# Autodesk Inventor assembly: Final Assembly
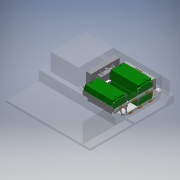
[picture p0: Inventor's stored thumbnail of the model, 180x180]
Saved by Autodesk Inventor 2017 (Build 210142000, 142)
## iProperties
Created: 2022-08-16
Part Number: Final Assembly
Document SubType Name: Assembly
Designer: JTS
Author: JTS
## Documents named in this file (24)
- G:\47 Ah FoMoCo Tray\02 Final Assembly (Tray Mated).iam
- G:\47 Ah FoMoCo Tray\LiBCM003 - Battery Tray\47 Ah FoMoCo Aluminum Tray.ipt
- G:\47 Ah FoMoCo Tray\OEM Parts\Junction Board.ipt
- G:\47 Ah FoMoCo Tray\OEM Parts\MCM.ipt
- G:\47 Ah FoMoCo Tray\Battery Modules\47Ah-FoMoCo.ipt
- G:\47 Ah FoMoCo Tray\LiBCM004 - Battery Rail\Bracket - 5th Module 8982K875.ipt
- G:\47 Ah FoMoCo Tray\Nuts & Bolts\Ring Terminal.ipt
- G:\47 Ah FoMoCo Tray\Final Assembly\AIP\Cable and Harness\Final Assembly.Harness2.iam
- G:\47 Ah FoMoCo Tray\LiBCM PCB\LiBCM Safety Cover - RevC.ipt
- G:\47 Ah FoMoCo Tray\LiBCM PCB\PCB.ipt
- G:\47 Ah FoMoCo Tray\OEM Parts\IMA Bay - Battery Enclosure Interface.ipt
- G:\47 Ah FoMoCo Tray\Nuts & Bolts\Battery Bolt.iam
- G:\47 Ah FoMoCo Tray\Nuts & Bolts\Threaded Standoff.ipt
- G:\47 Ah FoMoCo Tray\Nuts & Bolts\Battery Bolt - Split Washer.iam
- G:\47 Ah FoMoCo Tray\Nuts & Bolts\Washer 0.250in 92141A029.ipt
- G:\47 Ah FoMoCo Tray\Nuts & Bolts\Nut - Hex - 0.250in-20 91845A029.ipt
- G:\47 Ah FoMoCo Tray\Nuts & Bolts\Top Spacer.ipt
- G:\47 Ah FoMoCo Tray\Nuts & Bolts\PEMSERT.ipt
- G:\47 Ah FoMoCo Tray\Grid Chargers\UHP-1500-230.ipt
- G:\47 Ah FoMoCo Tray\Grid Chargers\HLG-480H-C2100B.ipt
- G:\47 Ah FoMoCo Tray\LiBCM005 - Charger Mount\Charger Mount.ipt
- G:\47 Ah FoMoCo Tray\Grid Chargers\HLG-240H-C1050B.ipt
- G:\47 Ah FoMoCo Tray\Nuts & Bolts\Fan.ipt
- G:\47 Ah FoMoCo Tray\Nuts & Bolts\Power Resistor - HSA25.ipt
## Components (86 placed, 23 different names)
1. IMA Bay - Battery Enclosure Interface:1 — Insert:56, Mate:2, Mate:3, Mate:4
2. Junction Board:1 — Insert:11, Insert:12
3. MCM:1 — Insert:137, Insert:138
4. Harness2 [sub-assembly]
5. Washer 0.250in 92141A029:3 — Insert:124
6. Nut - Hex - 0.250in-20 91845A029:5
7. Top Spacer:1 — Insert:125, Insert:126
8. PEMSERT:1 — Insert:129
9. PEMSERT:2 — Insert:130
10. PEMSERT:3 — Insert:131
11. PEMSERT:4 — Insert:132
12. UHP-1500-230:1 — Mate:5, Mate:6, Flush:2, Flush:8, Flush:9
13. HLG-240H-C1050B:1 — Mate:8, Flush:10, Flush:11
14. HLG-480H-C2100B:1 — Mate:7, Flush:8, Flush:9, Flush:10, Flush:11
15. Charger Mount:1 — Flush:5, Flush:6, Mate:8, Insert:133, Insert:134
16. Fan:1 — Insert:133, Insert:134
17. Power Resistor - HSA25:15 — Mate:9, Mate:10, Flush:16
18. Power Resistor - HSA25:11 — Mate:11, Flush:12, Flush:31
19. Power Resistor - HSA25:9 — Mate:12, Flush:27, Flush:28
20. Power Resistor - HSA25:12 — Mate:21, Flush:20
21. Power Resistor - HSA25:3 — Mate:23
22. Power Resistor - HSA25:10 — Mate:15, Flush:30, Flush:31
23. Power Resistor - HSA25:16 — Mate:16, Flush:16, Flush:17
24. Power Resistor - HSA25:17 — Mate:17, Flush:17, Flush:18
25. Power Resistor - HSA25:18 — Mate:18, Flush:18
26. Power Resistor - HSA25:13 — Mate:19, Mate:34, Mate:35
27. Power Resistor - HSA25:2 — Mate:24, Flush:23
28. Power Resistor - HSA25:5 — Mate:26, Flush:24
29. Power Resistor - HSA25:6 — Mate:32, Flush:24, Flush:25
30. Power Resistor - HSA25:4 — Mate:27, Flush:25
31. Power Resistor - HSA25:8 — Mate:28, Flush:26, Flush:27
32. Power Resistor - HSA25:7 — Mate:30, Mate:36, Flush:26
33. Power Resistor - HSA25:14 — Mate:31, Flush:29
34. Power Resistor - HSA25:1 — Mate:33, Flush:22
35. Power Resistor - HSA25:19 — Mate:37, Flush:28
36. Top Spacer:2 — Insert:135, Insert:138
37. Top Spacer:3 — Insert:136, Insert:137
38. Power Resistor - HSA25:20 — Mate:38, Flush:30
39. 47 Ah FoMoCo Aluminum Tray:1 — Insert:11, Insert:12, Insert:56, Mate:2, Insert:97, Insert:98, Insert:99, Insert:100, Insert:101, Insert:102, Insert:103, Insert:104, Insert:105, Insert:106, Insert:107, Insert:108, Insert:124, Mate:9, Mate:10, Mate:11, Flush:12, Mate:12, Mate:15, Mate:16, Mate:17, Mate:18, Mate:26, Mate:27, Mate:28, Mate:30, Mate:32, Mate:36, Mate:37, Insert:135, Insert:136, Mate:38
40. LiBCM Safety Cover - RevC:1 — Insert:55, Mate:1, Mate:3, Flush:1, Mate:4
41. PCB:1 — Insert:55, Mate:1
42. Threaded Standoff:1 — Insert:65
43. Threaded Standoff:2 — Insert:70
44. Threaded Standoff:3 — Insert:71
45. Threaded Standoff:4 — Insert:72, Insert:114
46. Threaded Standoff:5 — Insert:69, Insert:113
47. Threaded Standoff:6 — Insert:68, Insert:110
48. Threaded Standoff:7 — Insert:67
49. Threaded Standoff:8 — Insert:66, Insert:109
50. Battery Bolt:1 [sub-assembly] — Insert:102
51. Battery Bolt:2 [sub-assembly] — Insert:101
52. Battery Bolt:3 [sub-assembly] — Insert:99
53. Battery Bolt:4 [sub-assembly] — Insert:98
54. Battery Bolt:5 [sub-assembly] — Insert:100
55. Battery Bolt:6 [sub-assembly] — Insert:104
56. Battery Bolt:7 [sub-assembly] — Insert:103
57. Battery Bolt:8 [sub-assembly] — Insert:97
58. 47Ah-FoMoCo:1 — Insert:41, Insert:43, Tangent:1, Tangent:7, Insert:65, Insert:66, Insert:71, Insert:72, Insert:107, Insert:108
59. 47Ah-FoMoCo:2 — Insert:42, Insert:44, Tangent:3, Tangent:13, Insert:67, Insert:68, Insert:69, Insert:70, Insert:105, Insert:106
60. Bracket - 5th Module 8982K875:1 — Insert:109, Insert:110, Insert:120, Insert:121, Insert:122, Insert:131, Insert:132, Mate:5, Mate:6, Flush:2, Mate:7, Mate:19, Mate:21, Mate:31, Flush:20, Mate:34, Mate:35, Flush:29
61. Bracket - 5th Module 8982K875:2 — Insert:113, Insert:114, Insert:117, Insert:118, Insert:119, Insert:129, Insert:130, Flush:5, Flush:6, Mate:23, Mate:24, Mate:33, Flush:22, Flush:23
62. Battery Bolt:9 [sub-assembly] — Insert:127
63. Battery Bolt:10 [sub-assembly] — Insert:128
64. Battery Bolt - Split Washer:1 [sub-assembly] — Insert:77
65. Battery Bolt - Split Washer:2 [sub-assembly] — Insert:78
66. Battery Bolt - Split Washer:3 [sub-assembly] — Insert:79
67. Battery Bolt - Split Washer:4 [sub-assembly] — Insert:80
68. Battery Bolt - Split Washer:5 [sub-assembly] — Insert:84
69. Battery Bolt - Split Washer:6 [sub-assembly] — Insert:83
70. Battery Bolt - Split Washer:7 [sub-assembly] — Insert:82
71. Battery Bolt - Split Washer:8 [sub-assembly] — Insert:81
72. Battery Bolt - Split Washer:9 [sub-assembly] — Insert:126
73. Battery Bolt - Split Washer:10 [sub-assembly] — Insert:85
74. 47Ah-FoMoCo:3 — Insert:37, Insert:40, Tangent:9, Tangent:12, Flush:1, Insert:79, Insert:80, Insert:81, Insert:82, Insert:121, Insert:122
75. 47Ah-FoMoCo:4 — Insert:36, Insert:39, Tangent:14, Tangent:15, Insert:77, Insert:78, Insert:83, Insert:84, Insert:119, Insert:120
76. 47Ah-FoMoCo:5 — Insert:35, Insert:38, Tangent:16, Tangent:17, Insert:85, Insert:117, Insert:118, Insert:125, Insert:127, Insert:128
77. Ring Terminal:1 — Insert:35, Tangent:16
78. Ring Terminal:2 — Insert:36, Tangent:15
79. Ring Terminal:3 — Insert:37, Tangent:9
80. Ring Terminal:4 — Insert:38, Tangent:17
81. Ring Terminal:5 — Insert:39, Tangent:14
82. Ring Terminal:6 — Insert:40, Tangent:12
83. Ring Terminal:7 — Insert:41, Tangent:1
84. Ring Terminal:8 — Insert:42, Tangent:13
85. Ring Terminal:9 — Insert:43, Tangent:7
86. Ring Terminal:10 — Insert:44, Tangent:3
## Relationships (134: Insert 69, Mate 32, Flush 23, Tangent 10)
- Insert:11: Junction Board:1 ↔ 47 Ah FoMoCo Aluminum Tray:1
- Insert:12: Junction Board:1 ↔ 47 Ah FoMoCo Aluminum Tray:1
- Insert:35: 47Ah-FoMoCo:5 ↔ Ring Terminal:1
- Insert:36: 47Ah-FoMoCo:4 ↔ Ring Terminal:2
- Insert:37: 47Ah-FoMoCo:3 ↔ Ring Terminal:3
- Insert:38: 47Ah-FoMoCo:5 ↔ Ring Terminal:4
- Insert:39: 47Ah-FoMoCo:4 ↔ Ring Terminal:5
- Insert:40: 47Ah-FoMoCo:3 ↔ Ring Terminal:6
- Insert:41: 47Ah-FoMoCo:1 ↔ Ring Terminal:7
- Insert:42: 47Ah-FoMoCo:2 ↔ Ring Terminal:8
- Insert:43: 47Ah-FoMoCo:1 ↔ Ring Terminal:9
- Insert:44: 47Ah-FoMoCo:2 ↔ Ring Terminal:10
- Tangent:1 (2 mm): 47Ah-FoMoCo:1 ↔ Ring Terminal:7
- Tangent:3 (4 mm): 47Ah-FoMoCo:2 ↔ Ring Terminal:10
- Tangent:7 (6 mm): 47Ah-FoMoCo:1 ↔ Ring Terminal:9
- Tangent:9 (2 mm): 47Ah-FoMoCo:3 ↔ Ring Terminal:3
- Tangent:12 (2 mm): 47Ah-FoMoCo:3 ↔ Ring Terminal:6
- Tangent:13 (2 mm): 47Ah-FoMoCo:2 ↔ Ring Terminal:8
- Tangent:14 (2 mm): 47Ah-FoMoCo:4 ↔ Ring Terminal:5
- Tangent:15 (2 mm): 47Ah-FoMoCo:4 ↔ Ring Terminal:2
- Tangent:16 (2 mm): 47Ah-FoMoCo:5 ↔ Ring Terminal:1
- Tangent:17 (2 mm): 47Ah-FoMoCo:5 ↔ Ring Terminal:4
- Insert:55 (37 mm): LiBCM Safety Cover - RevC:1 ↔ PCB:1
- Mate:1: LiBCM Safety Cover - RevC:1 ↔ PCB:1
- Insert:56: IMA Bay - Battery Enclosure Interface:1 ↔ 47 Ah FoMoCo Aluminum Tray:1
- Mate:2: IMA Bay - Battery Enclosure Interface:1 ↔ 47 Ah FoMoCo Aluminum Tray:1
- Mate:3 (5 mm): IMA Bay - Battery Enclosure Interface:1 ↔ LiBCM Safety Cover - RevC:1
- Flush:1 (45 mm): LiBCM Safety Cover - RevC:1 ↔ 47Ah-FoMoCo:3
- Mate:4 (31.5 mm): IMA Bay - Battery Enclosure Interface:1 ↔ LiBCM Safety Cover - RevC:1
- Insert:65: Threaded Standoff:1 ↔ 47Ah-FoMoCo:1
- Insert:66: Threaded Standoff:8 ↔ 47Ah-FoMoCo:1
- Insert:67: Threaded Standoff:7 ↔ 47Ah-FoMoCo:2
- Insert:68: Threaded Standoff:6 ↔ 47Ah-FoMoCo:2
- Insert:69: Threaded Standoff:5 ↔ 47Ah-FoMoCo:2
- Insert:70: Threaded Standoff:2 ↔ 47Ah-FoMoCo:2
- Insert:71: Threaded Standoff:3 ↔ 47Ah-FoMoCo:1
- Insert:72: Threaded Standoff:4 ↔ 47Ah-FoMoCo:1
- Insert:77: Battery Bolt - Split Washer:1 ↔ 47Ah-FoMoCo:4
- Insert:78: Battery Bolt - Split Washer:2 ↔ 47Ah-FoMoCo:4
- Insert:79: Battery Bolt - Split Washer:3 ↔ 47Ah-FoMoCo:3
- Insert:80: Battery Bolt - Split Washer:4 ↔ 47Ah-FoMoCo:3
- Insert:81: Battery Bolt - Split Washer:8 ↔ 47Ah-FoMoCo:3
- Insert:82: Battery Bolt - Split Washer:7 ↔ 47Ah-FoMoCo:3
- Insert:83: Battery Bolt - Split Washer:6 ↔ 47Ah-FoMoCo:4
- Insert:84: Battery Bolt - Split Washer:5 ↔ 47Ah-FoMoCo:4
- Insert:85: Battery Bolt - Split Washer:10 ↔ 47Ah-FoMoCo:5
- Insert:97: 47 Ah FoMoCo Aluminum Tray:1 ↔ Battery Bolt:8
- Insert:98: 47 Ah FoMoCo Aluminum Tray:1 ↔ Battery Bolt:4
- Insert:99: 47 Ah FoMoCo Aluminum Tray:1 ↔ Battery Bolt:3
- Insert:100: 47 Ah FoMoCo Aluminum Tray:1 ↔ Battery Bolt:5
- Insert:101: 47 Ah FoMoCo Aluminum Tray:1 ↔ Battery Bolt:2
- Insert:102: 47 Ah FoMoCo Aluminum Tray:1 ↔ Battery Bolt:1
- Insert:103: 47 Ah FoMoCo Aluminum Tray:1 ↔ Battery Bolt:7
- Insert:104: 47 Ah FoMoCo Aluminum Tray:1 ↔ Battery Bolt:6
- Insert:105: 47 Ah FoMoCo Aluminum Tray:1 ↔ 47Ah-FoMoCo:2
- Insert:106: 47 Ah FoMoCo Aluminum Tray:1 ↔ 47Ah-FoMoCo:2
- Insert:107: 47 Ah FoMoCo Aluminum Tray:1 ↔ 47Ah-FoMoCo:1
- Insert:108: 47 Ah FoMoCo Aluminum Tray:1 ↔ 47Ah-FoMoCo:1
- Insert:109: Threaded Standoff:8 ↔ Bracket - 5th Module 8982K875:1
- Insert:110: Threaded Standoff:6 ↔ Bracket - 5th Module 8982K875:1
- Insert:113: Threaded Standoff:5 ↔ Bracket - 5th Module 8982K875:2
- Insert:114: Threaded Standoff:4 ↔ Bracket - 5th Module 8982K875:2
- Insert:117: Bracket - 5th Module 8982K875:2 ↔ 47Ah-FoMoCo:5
- Insert:118: Bracket - 5th Module 8982K875:2 ↔ 47Ah-FoMoCo:5
- Insert:119: Bracket - 5th Module 8982K875:2 ↔ 47Ah-FoMoCo:4
- Insert:120: Bracket - 5th Module 8982K875:1 ↔ 47Ah-FoMoCo:4
- Insert:121: Bracket - 5th Module 8982K875:1 ↔ 47Ah-FoMoCo:3
- Insert:122: Bracket - 5th Module 8982K875:1 ↔ 47Ah-FoMoCo:3
- [Insert]: Washer 0.250in 92141A029:3 ↔ Nut - Hex - 0.250in-20 91845A029:5
- Insert:124: Washer 0.250in 92141A029:3 ↔ 47 Ah FoMoCo Aluminum Tray:1
- Insert:125: Top Spacer:1 ↔ 47Ah-FoMoCo:5
- Insert:126: Top Spacer:1 ↔ Battery Bolt - Split Washer:9
- Insert:127: Battery Bolt:9 ↔ 47Ah-FoMoCo:5
- Insert:128: Battery Bolt:10 ↔ 47Ah-FoMoCo:5
- Insert:129: PEMSERT:1 ↔ Bracket - 5th Module 8982K875:2
- Insert:130: PEMSERT:2 ↔ Bracket - 5th Module 8982K875:2
- Insert:131: PEMSERT:3 ↔ Bracket - 5th Module 8982K875:1
- Insert:132: PEMSERT:4 ↔ Bracket - 5th Module 8982K875:1
- Mate:5: UHP-1500-230:1 ↔ Bracket - 5th Module 8982K875:1
- Mate:6 (1 mm): UHP-1500-230:1 ↔ Bracket - 5th Module 8982K875:1
- Flush:2: UHP-1500-230:1 ↔ Bracket - 5th Module 8982K875:1
- Mate:7: HLG-480H-C2100B:1 ↔ Bracket - 5th Module 8982K875:1
- Flush:5: Charger Mount:1 ↔ Bracket - 5th Module 8982K875:2
- Flush:6: Charger Mount:1 ↔ Bracket - 5th Module 8982K875:2
- Mate:8: HLG-240H-C1050B:1 ↔ Charger Mount:1
- Flush:8: UHP-1500-230:1 ↔ HLG-480H-C2100B:1
- Flush:9: UHP-1500-230:1 ↔ HLG-480H-C2100B:1
- Flush:10: HLG-240H-C1050B:1 ↔ HLG-480H-C2100B:1
- Flush:11: HLG-240H-C1050B:1 ↔ HLG-480H-C2100B:1
- Insert:133: Charger Mount:1 ↔ Fan:1
- Insert:134: Charger Mount:1 ↔ Fan:1
- Mate:9: Power Resistor - HSA25:15 ↔ 47 Ah FoMoCo Aluminum Tray:1
- Mate:10 (2.5 mm): Power Resistor - HSA25:15 ↔ 47 Ah FoMoCo Aluminum Tray:1
- Mate:11: Power Resistor - HSA25:11 ↔ 47 Ah FoMoCo Aluminum Tray:1
- Flush:12: Power Resistor - HSA25:11 ↔ 47 Ah FoMoCo Aluminum Tray:1
- Mate:12: Power Resistor - HSA25:9 ↔ 47 Ah FoMoCo Aluminum Tray:1
- Mate:15: Power Resistor - HSA25:10 ↔ 47 Ah FoMoCo Aluminum Tray:1
- Mate:16: Power Resistor - HSA25:16 ↔ 47 Ah FoMoCo Aluminum Tray:1
- Flush:16: Power Resistor - HSA25:15 ↔ Power Resistor - HSA25:16
- Mate:17: Power Resistor - HSA25:17 ↔ 47 Ah FoMoCo Aluminum Tray:1
- Flush:17: Power Resistor - HSA25:16 ↔ Power Resistor - HSA25:17
- Mate:18: Power Resistor - HSA25:18 ↔ 47 Ah FoMoCo Aluminum Tray:1
- Flush:18: Power Resistor - HSA25:17 ↔ Power Resistor - HSA25:18
- Mate:19: Power Resistor - HSA25:13 ↔ Bracket - 5th Module 8982K875:1
- Mate:21: Power Resistor - HSA25:12 ↔ Bracket - 5th Module 8982K875:1
- Mate:23: Power Resistor - HSA25:3 ↔ Bracket - 5th Module 8982K875:2
- Mate:24: Power Resistor - HSA25:2 ↔ Bracket - 5th Module 8982K875:2
- Mate:26: Power Resistor - HSA25:5 ↔ 47 Ah FoMoCo Aluminum Tray:1
- Mate:27: Power Resistor - HSA25:4 ↔ 47 Ah FoMoCo Aluminum Tray:1
- Mate:28: Power Resistor - HSA25:8 ↔ 47 Ah FoMoCo Aluminum Tray:1
- Mate:30: Power Resistor - HSA25:7 ↔ 47 Ah FoMoCo Aluminum Tray:1
- Mate:31: Power Resistor - HSA25:14 ↔ Bracket - 5th Module 8982K875:1
- Mate:32: Power Resistor - HSA25:6 ↔ 47 Ah FoMoCo Aluminum Tray:1
- Mate:33: Power Resistor - HSA25:1 ↔ Bracket - 5th Module 8982K875:2
- Flush:20: Power Resistor - HSA25:12 ↔ Bracket - 5th Module 8982K875:1
- Mate:34: Power Resistor - HSA25:13 ↔ Bracket - 5th Module 8982K875:1
- Mate:35: Power Resistor - HSA25:13 ↔ Bracket - 5th Module 8982K875:1
- Flush:22: Power Resistor - HSA25:1 ↔ Bracket - 5th Module 8982K875:2
- Flush:23: Power Resistor - HSA25:2 ↔ Bracket - 5th Module 8982K875:2
- Flush:24: Power Resistor - HSA25:5 ↔ Power Resistor - HSA25:6
- Flush:25: Power Resistor - HSA25:6 ↔ Power Resistor - HSA25:4
- Mate:36 (1 mm): Power Resistor - HSA25:7 ↔ 47 Ah FoMoCo Aluminum Tray:1
- Flush:26: Power Resistor - HSA25:8 ↔ Power Resistor - HSA25:7
- Flush:27: Power Resistor - HSA25:9 ↔ Power Resistor - HSA25:8
- Mate:37: Power Resistor - HSA25:19 ↔ 47 Ah FoMoCo Aluminum Tray:1
- Flush:28: Power Resistor - HSA25:9 ↔ Power Resistor - HSA25:19
- Flush:29: Power Resistor - HSA25:14 ↔ Bracket - 5th Module 8982K875:1
- Insert:135: Top Spacer:2 ↔ 47 Ah FoMoCo Aluminum Tray:1
- Insert:136: Top Spacer:3 ↔ 47 Ah FoMoCo Aluminum Tray:1
- Insert:137: MCM:1 ↔ Top Spacer:3
- Insert:138: MCM:1 ↔ Top Spacer:2
- Mate:38: Power Resistor - HSA25:20 ↔ 47 Ah FoMoCo Aluminum Tray:1
- Flush:30: Power Resistor - HSA25:10 ↔ Power Resistor - HSA25:20
- Flush:31: Power Resistor - HSA25:11 ↔ Power Resistor - HSA25:10
## Named parameters: d147_d115 = 0 mm
